# Autodesk Inventor assembly: prowadzenie2
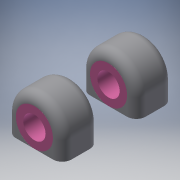
[picture p0: Inventor's stored thumbnail of the model, 180x180]
Saved by Autodesk Inventor 2019 (Build 230136000, 136)
## iProperties
Created: 2020-01-12
Part Number: prowadzenie2
Material: Ogólny
Document SubType Name: Assembly
Designer: Karolina
Author: Karolina
## Documents named in this file (3)
- C:\Users\Karolina\Desktop\Kuba\rekav2\dlon\prowadzenie2.iam
- C:\Users\Karolina\Desktop\Kuba\rekav2\dlon\trzym.ipt
- C:\Users\Karolina\Desktop\Kuba\rekav2\dlon\lozysko.ipt
## Components (4 placed, 2 different names)
1. trzym:1 — Zestawiający:1, Równoległy:2, Równoległy:3, Zestawiający:4
2. trzym:2 — Zestawiający:2, Równoległy:1, Równoległy:3, Zestawiający:4
3. lozysko:1 — Zestawiający:2, Równoległy:1, Zestawiający:3
4. lozysko:2 — Zestawiający:1, Równoległy:2, Zestawiający:3
## Relationships (7: Mate 4, Flush 3)
- Zestawiający:1 [Mate]: trzym:1 ↔ lozysko:2
- Zestawiający:2 [Mate]: trzym:2 ↔ lozysko:1
- Równoległy:1 [Flush]: trzym:2 ↔ lozysko:1
- Równoległy:2 [Flush]: trzym:1 ↔ lozysko:2
- Zestawiający:3 [Mate]: lozysko:1 ↔ lozysko:2
- Równoległy:3 [Flush]: trzym:1 ↔ trzym:2
- Zestawiający:4 [Mate] (1 mm): trzym:1 ↔ trzym:2
